# Autodesk Inventor assembly: POM_T5_01
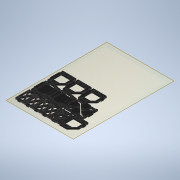
[picture p0: Inventor's stored thumbnail of the model, 180x180]
Saved by Autodesk Inventor 2020 (Build 240168000, 168)
## iProperties
Created: 2021-08-27
Part Number: POM_T5_01
Document SubType Name: Assembly
Designer: Masato
Author: Masato
## Documents named in this file (7)
- C:\Users\naoki\Documents\Inventor\CitBrains\git_clone\SUSTAINA_ver1_0\GFRP_2\SUSTAINA-OP\Cam\POM_T5_01.iam
- C:\Users\naoki\Documents\Inventor\CitBrains\git_clone\SUSTAINA_ver1_0\GFRP_2\SUSTAINA-OP\Cam\DisposableBoard.ipt
- C:\Users\naoki\Documents\Inventor\CitBrains\git_clone\SUSTAINA_ver1_0\GFRP_2\SUSTAINA-OP\UpperBody\Head\Camera_root_frame.ipt
- C:\Users\naoki\Documents\Inventor\CitBrains\git_clone\SUSTAINA_ver1_0\GFRP_2\SUSTAINA-OP\UpperBody\Head\Head_diagonal.ipt
- C:\Users\naoki\Documents\Inventor\CitBrains\git_clone\SUSTAINA_ver1_0\GFRP_2\SUSTAINA-OP\UpperBody\Head\Head_horn_frame.ipt
- C:\Users\naoki\Documents\Inventor\CitBrains\git_clone\SUSTAINA_ver1_0\GFRP_2\SUSTAINA-OP\UpperBody\Arm\ForeArm_diagonal.ipt
- C:\Users\naoki\Documents\Inventor\CitBrains\git_clone\SUSTAINA_ver1_0\GFRP_2\SUSTAINA-OP\UpperBody\Head\Camera_side_frame.ipt
## Components (16 placed, 6 different names)
1. DisposableBoard:1 — メイト:2, メイト:1, フラッシュ:1, フラッシュ:2, フラッシュ:3, フラッシュ:4, メイト:4, メイト:5, メイト:13, メイト:22, メイト:25, メイト:27, メイト:29, フラッシュ:12, フラッシュ:13, メイト:33, メイト:35, メイト:38, メイト:39
2. Camera_root_frame:1 — メイト:27, フラッシュ:11, メイト:41, メイト:48
3. Head_horn_frame:1 — メイト:29, フラッシュ:12, メイト:30, メイト:31, メイト:32
4. Camera_side_frame:1 — メイト:25, メイト:46, メイト:47, 正接:2
5. Camera_side_frame:2 — メイト:22, メイト:42, メイト:44, フラッシュ:14, メイト:47, メイト:52
6. ForeArm_diagonal:4 — フラッシュ:13, メイト:31, メイト:32, メイト:33, メイト:51
7. Camera_side_frame:3 — メイト:35, メイト:37, 正接:1, メイト:44, フラッシュ:14, メイト:51
8. Camera_side_frame:4 — メイト:37, 正接:1, メイト:38, メイト:46, 正接:2
9. Camera_root_frame:2 — メイト:39, メイト:41, メイト:42, メイト:49
10. Head_diagonal:2 — フラッシュ:3, フラッシュ:4, メイト:4, フラッシュ:5, メイト:6, フラッシュ:9, フラッシュ:11, メイト:48
11. Head_diagonal:1 — フラッシュ:5, メイト:5, メイト:6
12. Head_diagonal:3 — メイト:49
13. Head_diagonal:4 — メイト:30
14. ForeArm_diagonal:1 — メイト:13, フラッシュ:9
15. ForeArm_diagonal:5
16. ForeArm_diagonal:6 — メイト:52
## Component patterns: (2 elements, first: Head_diagonal:2 + Head_diagonal:1), (3 elements, first: ForeArm_diagonal:1)
## Relationships (39: Mate 27, Flush 10, Tangent 2)
- メイト:2 [Mate]: DisposableBoard:1
- メイト:1 [Mate]: DisposableBoard:1
- フラッシュ:1 [Flush]: DisposableBoard:1
- フラッシュ:2 [Flush]: DisposableBoard:1
- フラッシュ:3 [Flush] (2 mm): DisposableBoard:1 ↔ Head_diagonal:2
- フラッシュ:4 [Flush] (2 mm): DisposableBoard:1 ↔ Head_diagonal:2
- メイト:4 [Mate]: DisposableBoard:1 ↔ Head_diagonal:2
- フラッシュ:5 [Flush]: Head_diagonal:2 ↔ Head_diagonal:1
- メイト:5 [Mate]: DisposableBoard:1 ↔ Head_diagonal:1
- メイト:6 [Mate] (2.5 mm): Head_diagonal:2 ↔ Head_diagonal:1
- メイト:13 [Mate]: DisposableBoard:1 ↔ ForeArm_diagonal:1
- フラッシュ:9 [Flush]: Head_diagonal:2 ↔ ForeArm_diagonal:1
- メイト:22 [Mate]: DisposableBoard:1 ↔ Camera_side_frame:2
- メイト:25 [Mate]: DisposableBoard:1 ↔ Camera_side_frame:1
- メイト:27 [Mate]: DisposableBoard:1 ↔ Camera_root_frame:1
- フラッシュ:11 [Flush]: Camera_root_frame:1 ↔ Head_diagonal:2
- メイト:29 [Mate]: DisposableBoard:1 ↔ Head_horn_frame:1
- フラッシュ:12 [Flush] (2 mm): DisposableBoard:1 ↔ Head_horn_frame:1
- フラッシュ:13 [Flush] (2 mm): DisposableBoard:1 ↔ ForeArm_diagonal:4
- メイト:30 [Mate] (2.5 mm): Head_horn_frame:1 ↔ Head_diagonal:4
- メイト:31 [Mate] (2.5 mm): Head_horn_frame:1 ↔ ForeArm_diagonal:4
- メイト:32 [Mate] (2.5 mm): Head_horn_frame:1 ↔ ForeArm_diagonal:4
- メイト:33 [Mate]: DisposableBoard:1 ↔ ForeArm_diagonal:4
- メイト:35 [Mate]: DisposableBoard:1 ↔ Camera_side_frame:3
- メイト:37 [Mate] (2.5 mm): Camera_side_frame:3 ↔ Camera_side_frame:4
- 正接:1 [Tangent] (2.5 mm): Camera_side_frame:3 ↔ Camera_side_frame:4
- メイト:38 [Mate]: DisposableBoard:1 ↔ Camera_side_frame:4
- メイト:39 [Mate]: DisposableBoard:1 ↔ Camera_root_frame:2
- メイト:41 [Mate] (2.5 mm): Camera_root_frame:1 ↔ Camera_root_frame:2
- メイト:42 [Mate] (2.5 mm): Camera_side_frame:2 ↔ Camera_root_frame:2
- メイト:44 [Mate] (2.5 mm): Camera_side_frame:2 ↔ Camera_side_frame:3
- フラッシュ:14 [Flush]: Camera_side_frame:2 ↔ Camera_side_frame:3
- メイト:46 [Mate] (2.5 mm): Camera_side_frame:1 ↔ Camera_side_frame:4
- メイト:47 [Mate] (2.5 mm): Camera_side_frame:1 ↔ Camera_side_frame:2
- 正接:2 [Tangent] (2.5 mm): Camera_side_frame:1 ↔ Camera_side_frame:4
- メイト:48 [Mate] (2.5 mm): Camera_root_frame:1 ↔ Head_diagonal:2
- メイト:49 [Mate] (2.5 mm): Camera_root_frame:2 ↔ Head_diagonal:3
- メイト:51 [Mate] (2.5 mm): ForeArm_diagonal:4 ↔ Camera_side_frame:3
- メイト:52 [Mate] (2.5 mm): Camera_side_frame:2 ↔ ForeArm_diagonal:6
